# Autodesk Inventor assembly: sled
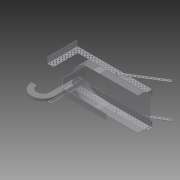
[picture p0: Inventor's stored thumbnail of the model, 180x180]
Saved by Autodesk Inventor 2014 SP1 (Build 180222100, 222)
## iProperties
Created: 2013-10-25
Part Number: sled
Document SubType Name: Assembly
Designer: RyanHughes
Author: RyanHughes
## Documents named in this file (13)
- C:\Users\Ryan\Desktop\sw\toss up 2ed A bot\intake\buckies poly\sled.iam
- C:\Users\Ryan\Desktop\sw\toss up 2ed A bot\intake\buckies poly\floor.ipt
- C:\Users\Ryan\Desktop\sw\lib\Aperture VEX CAD Library\Hardware\8-32\8-32_.375.ipt
- C:\Users\Ryan\Desktop\sw\toss up 2ed A bot\intake\buckies poly\side.ipt
- C:\Users\Ryan\Desktop\sw\toss up 2ed A bot\intake\buckies poly\back.ipt
- C:\Users\Ryan\Desktop\sw\lib\Aperture VEX CAD Library\Metal\Custom 1 bar\14 holes.ipt
- C:\Users\Ryan\Desktop\sw\lib\Aperture VEX CAD Library\Metal\L Bar\2 x 15.ipt
- C:\Users\Ryan\Desktop\sw\toss up 2ed A bot\intake\buckies poly\finger.ipt
- C:\Users\Ryan\Desktop\sw\lib\Aperture VEX CAD Library\Metal\L Bar\2 x 25.ipt
- C:\Users\Ryan\Desktop\sw\lib\Aperture VEX CAD Library\Metal\L Bar\2 x 10.ipt
- C:\Users\Ryan\Desktop\sw\toss up 2ed A bot\intake\buckies poly\hook.ipt
- C:\Users\Ryan\Desktop\sw\lib\Aperture VEX CAD Library\Linear Slide\Old version\Inside 5 hole.ipt
- C:\Users\Ryan\Desktop\sw\lib\Aperture VEX CAD Library\Linear Slide\Old version\Outside 5 hole.ipt
## Components (17 placed, 12 different names)
1. 2 x 15:1 — Flush:6, Flush:7, Mate:30, Mate:34, Mate:40, Mate:41, Flush:10, Flush:12, Mate:48
2. 2 x 15:2 — Flush:6, Flush:7, Mate:29, Mate:31, Mate:32, Mate:44, Mate:46, Mate:47
3. 8-32_.375:1 — Mate:20, Mate:21, Mate:38, Mate:40, Mate:48
4. 14 holes:1 — Mate:20, Mate:21, Mate:41, Angle:1
5. side:2 — Mate:18, Mate:32, Mate:33, Flush:8, Mate:37, Mate:45, Mate:51
6. back:1 — Mate:18, Mate:36, Mate:37, Tangent:1, Flush:11
7. floor:2 — Mate:29, Mate:30, Mate:31, Mate:33, Flush:8, Mate:35, Flush:9, Mate:36, Flush:10, Angle:2, Angle:3, Mate:49, Mate:52
8. side:3 — Mate:34, Mate:35, Flush:9, Mate:38, Mate:50, Flush:13
9. 8-32_.375:2 — Mate:45, Mate:46, Mate:47
10. 14 holes:2 — Mate:44, Angle:1
11. finger:1 — Tangent:1, Angle:2, Angle:3, Flush:11, Flush:12
12. 2 x 25:1 — Mate:49, Mate:50, Flush:13, Flush:14, Mate:53, Flush:15, Flush:16
13. 2 x 25:2 — Mate:51, Mate:52, Flush:14, Mate:54, Flush:17, Flush:18, Flush:19
14. 2 x 10:1 — Mate:53, Flush:15, Flush:16
15. hook:1 — Mate:55, Mate:57, Mate:58, Mate:59
16. Inside 5 hole:1 — Mate:54, Flush:17, Flush:18, Mate:56
17. Outside 5 hole:1 — Mate:55, Mate:56, Flush:19, Mate:57, Mate:58, Mate:59
## Relationships (51: Mate 33, Flush 14, Angle 3, Tangent 1)
- Mate:18: side:2 ↔ back:1
- Mate:20 (2.3114 mm): 8-32_.375:1 ↔ 14 holes:1
- Mate:21 (2.3114 mm): 8-32_.375:1 ↔ 14 holes:1
- Flush:6: 2 x 15:1 ↔ 2 x 15:2
- Flush:7: 2 x 15:1 ↔ 2 x 15:2
- Mate:29: 2 x 15:2 ↔ floor:2
- Mate:30: 2 x 15:1 ↔ floor:2
- Mate:31: 2 x 15:2 ↔ floor:2
- Mate:32: 2 x 15:2 ↔ side:2
- Mate:33: side:2 ↔ floor:2
- Flush:8: side:2 ↔ floor:2
- Mate:34: 2 x 15:1 ↔ side:3
- Mate:35: floor:2 ↔ side:3
- Flush:9: floor:2 ↔ side:3
- Mate:36: back:1 ↔ floor:2
- Mate:37 (-25.4 mm): side:2 ↔ back:1
- Mate:38: 8-32_.375:1 ↔ side:3
- Mate:40 (2.3114 mm): 2 x 15:1 ↔ 8-32_.375:1
- Mate:41: 2 x 15:1 ↔ 14 holes:1
- Flush:10 (1.27 mm): 2 x 15:1 ↔ floor:2
- [Mate] (2.3114 mm): 8-32_.375:2 ↔ 14 holes:2
- [Mate] (2.3114 mm): 8-32_.375:2 ↔ 14 holes:2
- Mate:44: 2 x 15:2 ↔ 14 holes:2
- Mate:45: side:2 ↔ 8-32_.375:2
- Mate:46 (2.3114 mm): 2 x 15:2 ↔ 8-32_.375:2
- Mate:47 (2.3114 mm): 2 x 15:2 ↔ 8-32_.375:2
- Angle:1 (0 deg): 14 holes:1 ↔ 14 holes:2
- Tangent:1: back:1 ↔ finger:1
- Angle:2 (180 deg): floor:2 ↔ finger:1
- Angle:3 (180 deg): floor:2 ↔ finger:1
- Flush:11: back:1 ↔ finger:1
- Flush:12 (-58.3184 mm): 2 x 15:1 ↔ finger:1
- Mate:48 (2.3114 mm): 2 x 15:1 ↔ 8-32_.375:1
- Mate:49: floor:2 ↔ 2 x 25:1
- Mate:50: side:3 ↔ 2 x 25:1
- Flush:13 (1.27 mm): side:3 ↔ 2 x 25:1
- Mate:51: side:2 ↔ 2 x 25:2
- Mate:52: floor:2 ↔ 2 x 25:2
- Flush:14: 2 x 25:1 ↔ 2 x 25:2
- Mate:53: 2 x 25:1 ↔ 2 x 10:1
- Flush:15: 2 x 25:1 ↔ 2 x 10:1
- Flush:16: 2 x 25:1 ↔ 2 x 10:1
- Mate:54: 2 x 25:2 ↔ Inside 5 hole:1
- Flush:17: 2 x 25:2 ↔ Inside 5 hole:1
- Flush:18: 2 x 25:2 ↔ Inside 5 hole:1
- Mate:55: hook:1 ↔ Outside 5 hole:1
- Mate:56 (10.16 mm): Inside 5 hole:1 ↔ Outside 5 hole:1
- Flush:19: 2 x 25:2 ↔ Outside 5 hole:1
- Mate:57 (2.3114 mm): hook:1 ↔ Outside 5 hole:1
- Mate:58 (2.3114 mm): hook:1 ↔ Outside 5 hole:1
- Mate:59 (2.3114 mm): hook:1 ↔ Outside 5 hole:1
## Named parameters: q = 2.3114 mm, d53_q = 2.3114 mm, d54_d25 = 2.3114 mm, d55_d26 = 2.3114 mm
